# Autodesk Inventor assembly: 20-J2
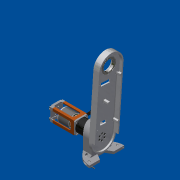
[picture p0: Inventor's stored thumbnail of the model, 180x180]
Saved by Autodesk Inventor 2018 (Build 220112000, 112)
## iProperties
Created: 2020-01-14
Part Number: 20-J2
Document SubType Name: Assembly
Designer: Bunny320
Author: Bunny320
## Documents named in this file (11)
- C:\Users\Bunny320\Desktop\sechs\4-CAD\20-J2.iam
- C:\Users\Bunny320\Desktop\sechs\4-CAD\201-flange-with motor.ipt
- C:\Users\Bunny320\Desktop\sechs\4-CAD\standardParts\61807-2RS1\61807-2RS1.iam
- C:\Users\Bunny320\Desktop\sechs\4-CAD\motor unit.iam
- C:\Users\Bunny320\Desktop\sechs\4-CAD\203-link left.ipt
- C:\Users\Bunny320\Documents\Inventor\Content Center Files\R2018\en-US\ISO 10642(2)\ISO 10642  - M4  x  20.ipt
- C:\Users\Bunny320\Documents\Inventor\Content Center Files\R2018\en-US\ISO 4762(1)\DIN EN ISO 4762 - M3 x 12.ipt
- C:\Users\Bunny320\Documents\Inventor\Content Center Files\R2018\en-US\ISO 4762(1)\DIN EN ISO 4762 - M3 x 20.ipt
- C:\Users\Bunny320\Documents\Inventor\Content Center Files\R2018\en-US\DIN EN ISO 4032\DIN EN ISO 4032 - M3.ipt
- C:\Users\Bunny320\Desktop\sechs\4-CAD\standardParts\Pololu mounting hub\pololu-universal-aluminum-mounting-hub-for-8mm-shaft-m3-holes.ipt
- C:\Users\Bunny320\Documents\Inventor\Content Center Files\R2018\en-US\ISO 10642(2)\ISO 10642  - M3  x  12.ipt
## Components (22 placed, 10 different names)
1. 201-flange-with motor:1 — Flush:1, Flush:2, Flush:3, Mate:3, Mate:7, Mate:8, Mate:9, Mate:21, Mate:22, Mate:23, Mate:24, Mate:31, Mate:32, Mate:33, Mate:34, Mate:35, Mate:36, Mate:37, Mate:38, Mate:39, Mate:40, Mate:41, Mate:42, Mate:48
2. 61807-2RS1:1 [sub-assembly] — Mate:3, Mate:14, Mate:45, Mate:48
3. motor unit:1 [sub-assembly] — Mate:7, Mate:8, Mate:9
4. 203-link left:1 — Mate:14, Mate:15, Mate:16, Mate:44, Mate:45, Mate:46, Mate:47, Mate:49, Mate:50, Mate:51, Mate:52, Mate:53, Mate:54
5. 61807-2RS1:3 [sub-assembly] — Mate:15, Mate:16
6. DIN EN ISO 10642 M4  x  20:1 — Mate:21
7. DIN EN ISO 10642 M4  x  20:2 — Mate:22
8. DIN EN ISO 10642 M4  x  20:3 — Mate:23
9. DIN EN ISO 10642 M4  x  20:4 — Mate:24
10. DIN EN ISO 4762 M3 x 12:4 — Mate:31, Mate:32
11. DIN EN ISO 4762 M3 x 12:5 — Mate:33, Mate:34
12. DIN EN ISO 4762 M3 x 12:6 — Mate:35, Mate:36
13. DIN EN ISO 4762 M3 x 12:7 — Mate:37, Mate:38
14. DIN EN ISO 4762 M3 x 20:1 — Mate:39, Mate:40
15. DIN EN ISO 4032 M3:1 — Mate:41, Mate:42
16. pololu-universal-aluminum-mounting-hub-for-8mm-shaft-m3-holes:1 — Mate:44, Mate:46, Mate:47
17. DIN EN ISO 10642 M3  x  12:1 — Mate:49
18. DIN EN ISO 10642 M3  x  12:2 — Mate:50
19. DIN EN ISO 10642 M3  x  12:3 — Mate:51
20. DIN EN ISO 10642 M3  x  12:4 — Mate:52
21. DIN EN ISO 10642 M3  x  12:5 — Mate:53
22. DIN EN ISO 10642 M3  x  12:6 — Mate:54
## Relationships (37: Mate 34, Flush 3)
- Flush:1: 201-flange-with motor:1
- Flush:2: 201-flange-with motor:1
- Flush:3: 201-flange-with motor:1
- Mate:3: 201-flange-with motor:1 ↔ 61807-2RS1:1
- Mate:7: 201-flange-with motor:1 ↔ motor unit:1
- Mate:8: 201-flange-with motor:1 ↔ motor unit:1
- Mate:9: 201-flange-with motor:1 ↔ motor unit:1
- Mate:14: 61807-2RS1:1 ↔ 203-link left:1
- Mate:15: 203-link left:1 ↔ 61807-2RS1:3
- Mate:16: 203-link left:1 ↔ 61807-2RS1:3
- Mate:21: 201-flange-with motor:1 ↔ DIN EN ISO 10642 M4  x  20:1
- Mate:22: 201-flange-with motor:1 ↔ DIN EN ISO 10642 M4  x  20:2
- Mate:23: 201-flange-with motor:1 ↔ DIN EN ISO 10642 M4  x  20:3
- Mate:24: 201-flange-with motor:1 ↔ DIN EN ISO 10642 M4  x  20:4
- Mate:31: 201-flange-with motor:1 ↔ DIN EN ISO 4762 M3 x 12:4
- Mate:32: 201-flange-with motor:1 ↔ DIN EN ISO 4762 M3 x 12:4
- Mate:33: 201-flange-with motor:1 ↔ DIN EN ISO 4762 M3 x 12:5
- Mate:34: 201-flange-with motor:1 ↔ DIN EN ISO 4762 M3 x 12:5
- Mate:35: 201-flange-with motor:1 ↔ DIN EN ISO 4762 M3 x 12:6
- Mate:36: 201-flange-with motor:1 ↔ DIN EN ISO 4762 M3 x 12:6
- Mate:37: 201-flange-with motor:1 ↔ DIN EN ISO 4762 M3 x 12:7
- Mate:38: 201-flange-with motor:1 ↔ DIN EN ISO 4762 M3 x 12:7
- Mate:39: 201-flange-with motor:1 ↔ DIN EN ISO 4762 M3 x 20:1
- Mate:40: 201-flange-with motor:1 ↔ DIN EN ISO 4762 M3 x 20:1
- Mate:41: 201-flange-with motor:1 ↔ DIN EN ISO 4032 M3:1
- Mate:42: 201-flange-with motor:1 ↔ DIN EN ISO 4032 M3:1
- Mate:44: 203-link left:1 ↔ pololu-universal-aluminum-mounting-hub-for-8mm-shaft-m3-holes:1
- Mate:45: 61807-2RS1:1 ↔ 203-link left:1
- Mate:46: 203-link left:1 ↔ pololu-universal-aluminum-mounting-hub-for-8mm-shaft-m3-holes:1
- Mate:47: 203-link left:1 ↔ pololu-universal-aluminum-mounting-hub-for-8mm-shaft-m3-holes:1
- Mate:48: 201-flange-with motor:1 ↔ 61807-2RS1:1
- Mate:49: 203-link left:1 ↔ DIN EN ISO 10642 M3  x  12:1
- Mate:50: 203-link left:1 ↔ DIN EN ISO 10642 M3  x  12:2
- Mate:51: 203-link left:1 ↔ DIN EN ISO 10642 M3  x  12:3
- Mate:52: 203-link left:1 ↔ DIN EN ISO 10642 M3  x  12:4
- Mate:53: 203-link left:1 ↔ DIN EN ISO 10642 M3  x  12:5
- Mate:54: 203-link left:1 ↔ DIN EN ISO 10642 M3  x  12:6
